# Autodesk Inventor assembly: SHOULDER
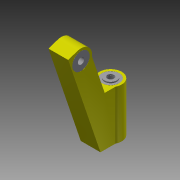
[picture p0: Inventor's stored thumbnail of the model, 180x180]
Saved by Autodesk Inventor 2013 (Build 170138000, 138)
## iProperties
Created: 2013-11-26
Part Number: SHOULDER
Document SubType Name: Assembly
Designer: employee
Author: employee
## Documents named in this file (4)
- C:\Users\employee\Desktop\GUS Simpson\SHOULDER.iam
- C:\Users\employee\Desktop\GUS Simpson\SHOULDER.ipt
- C:\Users\employee\Desktop\GUS Simpson\_608.ipt
- C:\Users\employee\Desktop\GUS Simpson\M8 WASHER.ipt
## Components (7 placed, 3 different names)
1. SHOULDER:1 — Insert:1, Insert:2, Insert:3, Insert:4
2. _608:1 — Insert:1
3. _608:2 — Insert:2
4. _608:3 — Insert:3, Insert:6
5. _608:4 — Insert:4, Insert:7
6. M8 WASHER:2 — Insert:6
7. M8 WASHER:3 — Insert:7
## Relationships (6: Insert 6)
- Insert:1: SHOULDER:1 ↔ _608:1
- Insert:2: SHOULDER:1 ↔ _608:2
- Insert:3: SHOULDER:1 ↔ _608:3
- Insert:4: SHOULDER:1 ↔ _608:4
- Insert:6: _608:3 ↔ M8 WASHER:2
- Insert:7: _608:4 ↔ M8 WASHER:3
